# Autodesk Inventor assembly: Galvo_Galvo_Tilted
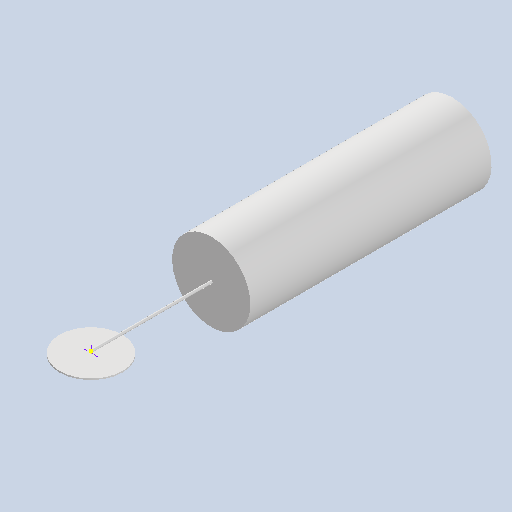
[picture p0: Inventor's stored thumbnail of the model, 512x512]
Saved by Autodesk Inventor 2025.2 (Build 292293000, 293)
## iProperties
Created: 2023-10-20
Part Number: Galvo_Galvo_Tilted
Document SubType Name: Assembly
Designer: S227943
Author: S227943
## Documents named in this file (2)
- C:\Users\monolithic\Documents\GitHub\CAD\Monolith\John\Altair_PowellBaseplate_SPIM_ASLM_CTASLM\Assembly\SubAssemblies\Galvo_Galvo_Tilted.iam
- C:\Users\monolithic\Documents\GitHub\CAD\Monolith\John\Altair_PowellBaseplate_SPIM_ASLM_CTASLM\Assembly\SubAssemblies\CRS4kHz.ipt
## Components (1 placed, 1 different names)
1. CRS4kHz:2 — Mate:1, Angle:1, Symmetry:1, Flush:1, Mate:2, Angle:2, Symmetry:2, Mate:3, Flush:2
## Relationships (10: Mate 3, Angle 3, Symmetry 2, Flush 2)
- Mate:1: CRS4kHz:2
- Angle:1 (90 deg): CRS4kHz:2
- Symmetry:1: CRS4kHz:2
- Flush:1: CRS4kHz:2
- Mate:2: CRS4kHz:2
- Angle:2 (0 deg): CRS4kHz:2
- Symmetry:2: CRS4kHz:2
- Mate:3: CRS4kHz:2
- Angle:3 (0 deg)
- Flush:2: CRS4kHz:2
